# Autodesk Inventor assembly: nc_nhk16
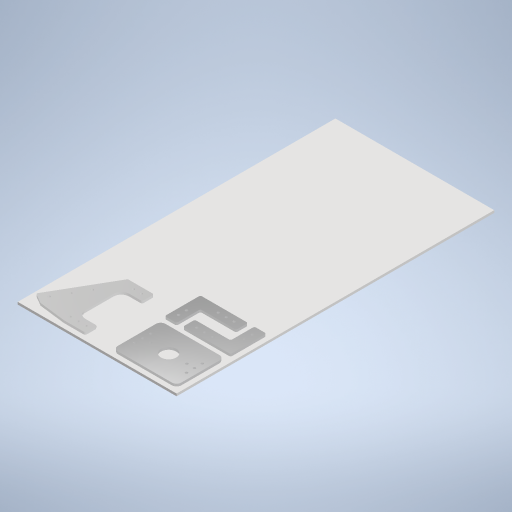
[picture p0: Inventor's stored thumbnail of the model, 512x512]
Saved by Autodesk Inventor 2023 (Build 270158000, 158)
## iProperties
Created: 2022-04-24
Part Number: nc_nhk16
Document SubType Name: Assembly
Designer: yuta
Author: yuta
## Documents named in this file (5)
- C:\Users\yuta\Documents\NHK\nc_nhk16.iam
- C:\Users\yuta\Documents\NHK\旧\NC.port.ipt
- C:\Users\yuta\Desktop\オムニホイール\ホイールユニット_側板1.ipt
- C:\Users\yuta\Documents\NHK\射出_エンコーダー固定2.ipt
- C:\Users\yuta\Documents\NHK\射出_固定6.ipt
## Components (5 placed, 4 different names)
1. NC.port:1 — メイト:1, フラッシュ:1, メイト:3, メイト:4, フラッシュ:2, フラッシュ:3, メイト:5, フラッシュ:4, メイト:7
2. ホイールユニット_側板1:1 — メイト:1, フラッシュ:1, メイト:3
3. 射出_エンコーダー固定2:1 — メイト:4, フラッシュ:2, フラッシュ:3, メイト:6, メイト:9
4. 射出_固定6:1 — メイト:5, フラッシュ:4, メイト:6, メイト:8
5. 射出_固定6:2 — メイト:7, メイト:8, メイト:9
## Relationships (12: Mate 8, Flush 4)
- メイト:1 [Mate]: NC.port:1 ↔ ホイールユニット_側板1:1
- フラッシュ:1 [Flush] (6 mm): NC.port:1 ↔ ホイールユニット_側板1:1
- メイト:3 [Mate] (-8 mm): NC.port:1 ↔ ホイールユニット_側板1:1
- メイト:4 [Mate]: NC.port:1 ↔ 射出_エンコーダー固定2:1
- フラッシュ:2 [Flush] (6 mm): NC.port:1 ↔ 射出_エンコーダー固定2:1
- フラッシュ:3 [Flush] (6 mm): NC.port:1 ↔ 射出_エンコーダー固定2:1
- メイト:5 [Mate]: NC.port:1 ↔ 射出_固定6:1
- フラッシュ:4 [Flush] (6 mm): NC.port:1 ↔ 射出_固定6:1
- メイト:6 [Mate] (8 mm): 射出_エンコーダー固定2:1 ↔ 射出_固定6:1
- メイト:7 [Mate]: NC.port:1 ↔ 射出_固定6:2
- メイト:8 [Mate] (8 mm): 射出_固定6:1 ↔ 射出_固定6:2
- メイト:9 [Mate] (8 mm): 射出_エンコーダー固定2:1 ↔ 射出_固定6:2
